# Autodesk Inventor assembly: TeflonHolder
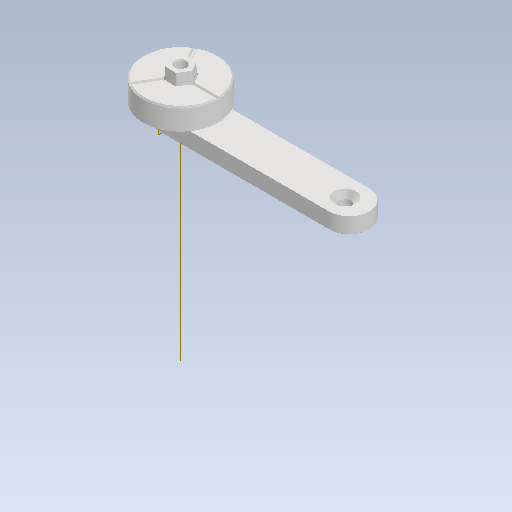
[picture p0: Inventor's stored thumbnail of the model, 512x512]
Saved by Autodesk Inventor 2020.3 (Build 243373010, 373A)
## iProperties
Created: 2020-01-17
Part Number: TeflonHolder
Document SubType Name: Assembly
Designer: Parker
Author: Parker
## Documents named in this file (4)
- D:\Designs\MK3PRO P1\ACCESSORIES\Teflon Holder\TeflonHolder.iam
- D:\Designs\MK3PRO P1\ACCESSORIES\Teflon Holder\TeflonHolder.ipt
- D:\Designs\MK3PRO P1\ACCESSORIES\Teflon Holder\TeflonHolderWasher.ipt
- D:\Designs\MK3PRO P1\ACCESSORIES\Teflon Holder\TeflonHolderNut.ipt
## Components (3 placed, 3 different names)
1. TeflonHolder:1 — Mate:1, Mate:2
2. TeflonHolderWasher:1 — Mate:1, Mate:2, Mate:3, Mate:4, Angle:1
3. TeflonHolderNut:1 — Mate:3, Mate:4, Angle:1
## Relationships (5: Mate 4, Angle 1)
- Mate:1: TeflonHolder:1 ↔ TeflonHolderWasher:1
- Mate:2: TeflonHolder:1 ↔ TeflonHolderWasher:1
- Mate:3: TeflonHolderWasher:1 ↔ TeflonHolderNut:1
- Mate:4: TeflonHolderWasher:1 ↔ TeflonHolderNut:1
- Angle:1 (0 deg): TeflonHolderWasher:1 ↔ TeflonHolderNut:1
